# Autodesk Inventor assembly: Z Motor Unit A
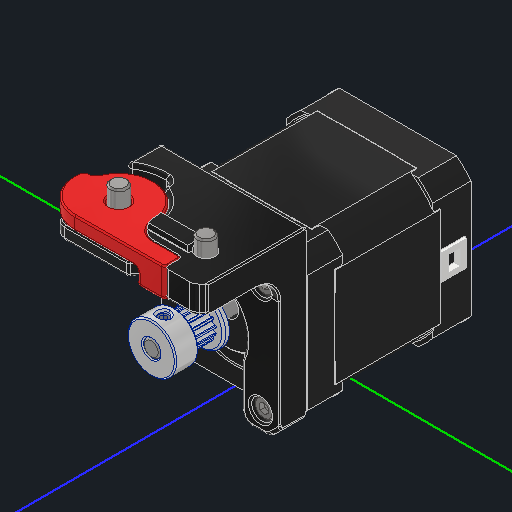
[picture p0: Inventor's stored thumbnail of the model, 512x512]
Saved by Autodesk Inventor 2022.2 (Build 262287010, 287A)
## iProperties
Created: 2022-03-12
Part Number: Z Motor Unit A
Document SubType Name: Assembly
Designer: sleib
Author: sleib
## Documents named in this file (7)
- C:\Users\sleib\Projekte\Voron-2\CAD\Inventor\Z Motor-Unit [A].iam
- C:\Users\sleib\Projekte\Voron-2\CAD\Inventor\NEMA17 Black.ipt
- C:\Users\sleib\Projekte\Voron-2\CAD\Inventor\GT2 16T Pulley (6mm).ipt
- C:\Users\sleib\Projekte\Voron-2\CAD\Inventor\Z Motor-Mount [A].ipt
- C:\Users\sleib\Projekte\Voron-2\CAD\Inventor\Z Belt-Tensioner [A].ipt
- C:\Users\sleib\Projekte\Voron-2\CAD\Inventor\M3x8 SHCS.ipt
- C:\Users\sleib\Projekte\Voron-2\CAD\Inventor\M5x10 BHCS.ipt
## Components (9 placed, 6 different names)
1. NEMA17 Black:1 — Passend:1, Fluchtend:1, Passend:7, Passend:8, Passend:9, Passend:18, Passend:19, Passend:24
2. GT2 16T Pulley (6mm):1 — Passend:1, Fluchtend:1
3. Z Motor-Mount [A]:1 — Passend:24, Passend:21, Passend:22, Passend:23, Passend:10, Passend:11, Passend:12, Passend:5, Passend:25, Passend:26, Passend:27, Passend:28
4. Z Belt-Tensioner [A]:1 — Passend:5, Passend:29
5. M3x8 SHCS:1 — Passend:7, Passend:12, Passend:18, Passend:21
6. M3x8 SHCS:2 — Passend:8, Passend:11, Passend:22
7. M3x8 SHCS:3 — Passend:9, Passend:23, Passend:10, Passend:19
8. M5x10 BHCS:2 — Passend:25, Passend:28, Passend:29
9. M5x10 BHCS:3 — Passend:26, Passend:27
## Relationships (20: Mate 19, Flush 1)
- Passend:1 [Mate]: NEMA17 Black:1 ↔ GT2 16T Pulley (6mm):1
- Fluchtend:1 [Flush]: NEMA17 Black:1 ↔ GT2 16T Pulley (6mm):1
- Passend:7 [Mate]: NEMA17 Black:1 ↔ M3x8 SHCS:1
- Passend:8 [Mate]: NEMA17 Black:1 ↔ M3x8 SHCS:2
- Passend:9 [Mate]: NEMA17 Black:1 ↔ M3x8 SHCS:3
- Passend:24 [Mate]: NEMA17 Black:1 ↔ Z Motor-Mount [A]:1
- Passend:21 [Mate]: Z Motor-Mount [A]:1 ↔ M3x8 SHCS:1
- Passend:22 [Mate]: Z Motor-Mount [A]:1 ↔ M3x8 SHCS:2
- Passend:23 [Mate]: Z Motor-Mount [A]:1 ↔ M3x8 SHCS:3
- Passend:10 [Mate]: Z Motor-Mount [A]:1 ↔ M3x8 SHCS:3
- Passend:11 [Mate]: Z Motor-Mount [A]:1 ↔ M3x8 SHCS:2
- Passend:12 [Mate]: Z Motor-Mount [A]:1 ↔ M3x8 SHCS:1
- Passend:18 [Mate]: NEMA17 Black:1 ↔ M3x8 SHCS:1
- Passend:19 [Mate]: NEMA17 Black:1 ↔ M3x8 SHCS:3
- Passend:5 [Mate]: Z Motor-Mount [A]:1 ↔ Z Belt-Tensioner [A]:1
- Passend:25 [Mate]: Z Motor-Mount [A]:1 ↔ M5x10 BHCS:2
- Passend:26 [Mate]: Z Motor-Mount [A]:1 ↔ M5x10 BHCS:3
- Passend:27 [Mate]: Z Motor-Mount [A]:1 ↔ M5x10 BHCS:3
- Passend:28 [Mate]: Z Motor-Mount [A]:1 ↔ M5x10 BHCS:2
- Passend:29 [Mate]: Z Belt-Tensioner [A]:1 ↔ M5x10 BHCS:2
